# Autodesk Inventor assembly: RP_ROBOT
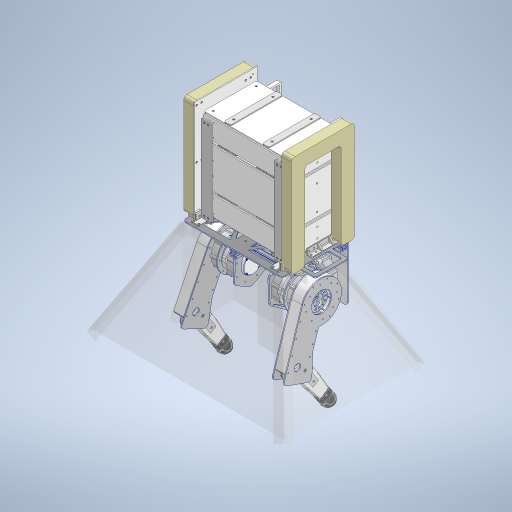
[picture p0: Inventor's stored thumbnail of the model, 512x512]
Saved by Autodesk Inventor 2024.3 (Build 283343000, 343)
## iProperties
Created: 2025-10-10
Part Number: RP_ROBOT
Document SubType Name: Assembly
Designer: 佐藤智貴
Mass: 38781.7 g
Surface Area: 40547 cm^2
Volume: 35004.9 cm^3
Density: 1.10789 g/cm^3
Author: 佐藤智貴
## Documents named in this file (34)
- C:\Users\佐藤智貴\OneDrive - Chiba Institute of Technology\ドキュメント\Inventor\Biped_Robot2\RP_ROBOT.iam
- C:\Users\佐藤智貴\OneDrive - Chiba Institute of Technology\ドキュメント\Inventor\Biped_Robot2\RP_Calf-Foot.ipt
- C:\Users\佐藤智貴\OneDrive - Chiba Institute of Technology\ドキュメント\Inventor\Biped_Robot2\RP_Calf-Link.ipt
- C:\Users\佐藤智貴\OneDrive - Chiba Institute of Technology\ドキュメント\Inventor\Biped_Robot2\RP_Waist-Under-ver2.ipt
- C:\Users\佐藤智貴\OneDrive - Chiba Institute of Technology\ドキュメント\Inventor\Biped_Robot2\RP_Waist-Avobe-ver2.ipt
- C:\Users\佐藤智貴\OneDrive - Chiba Institute of Technology\ドキュメント\Inventor\Biped_Robot2\CAF5-2020-140.ipt
- C:\Users\佐藤智貴\OneDrive - Chiba Institute of Technology\ドキュメント\Inventor\Biped_Robot2\CAF5-2020-170.ipt
- C:\Users\佐藤智貴\OneDrive - Chiba Institute of Technology\ドキュメント\Inventor\Biped_Robot2\CAF5-2020-175.ipt
- C:\Users\佐藤智貴\OneDrive - Chiba Institute of Technology\ドキュメント\Inventor\Biped_Robot2\HFBL45A5-2020-140.iam
- C:\Users\佐藤智貴\OneDrive - Chiba Institute of Technology\ドキュメント\Inventor\Biped_Robot2\8108-8.iam
- C:\Users\佐藤智貴\OneDrive - Chiba Institute of Technology\ドキュメント\Inventor\Biped_Robot2\RP_Hip-Base.ipt
- C:\Users\佐藤智貴\OneDrive - Chiba Institute of Technology\ドキュメント\Inventor\Biped_Robot2\RP_Hip-Link-Left.ipt
- C:\Users\佐藤智貴\OneDrive - Chiba Institute of Technology\ドキュメント\Inventor\Biped_Robot2\RP_Hip-Link-Right.ipt
- C:\Users\佐藤智貴\OneDrive - Chiba Institute of Technology\ドキュメント\Inventor\Biped_Robot2\RP_Calf-Link-cover-Inside-Left.ipt
- C:\Users\佐藤智貴\OneDrive - Chiba Institute of Technology\ドキュメント\Inventor\Biped_Robot2\RP_Calf-Link-cover-Inside-Right.ipt
- C:\Users\佐藤智貴\OneDrive - Chiba Institute of Technology\ドキュメント\Inventor\Biped_Robot2\RP_Calf-Link-cover-Outside-Left.ipt
- C:\Users\佐藤智貴\OneDrive - Chiba Institute of Technology\ドキュメント\Inventor\Biped_Robot2\RP_Calf-Link-cover-Outside-Right.ipt
- C:\Users\佐藤智貴\OneDrive - Chiba Institute of Technology\ドキュメント\Inventor\Biped_Robot2\RP_Thigh-Base_Left.ipt
- C:\Users\佐藤智貴\OneDrive - Chiba Institute of Technology\ドキュメント\Inventor\Biped_Robot2\RP_Thigh-Base-Cover.ipt
- C:\Users\佐藤智貴\OneDrive - Chiba Institute of Technology\ドキュメント\Inventor\Biped_Robot2\RP_Thigh-Base-Right.ipt
- C:\Users\佐藤智貴\OneDrive - Chiba Institute of Technology\ドキュメント\Inventor\Biped_Robot2\RP_Thigh-cover.ipt
- C:\Users\佐藤智貴\OneDrive - Chiba Institute of Technology\ドキュメント\Inventor\Biped_Robot2\RP_Thigh-cover-connect.ipt
- C:\Users\佐藤智貴\OneDrive - Chiba Institute of Technology\ドキュメント\Inventor\Biped_Robot2\RP_Thigh-Link.ipt
- C:\Users\佐藤智貴\OneDrive - Chiba Institute of Technology\ドキュメント\Inventor\Biped_Robot2\simring_34mm.ipt
- C:\Users\佐藤智貴\OneDrive - Chiba Institute of Technology\ドキュメント\Inventor\Biped_Robot2\F688ZZ.ipt
- C:\Users\佐藤智貴\OneDrive - Chiba Institute of Technology\ドキュメント\Inventor\Biped_Robot2\628ZZ.ipt
- C:\Users\佐藤智貴\OneDrive - Chiba Institute of Technology\ドキュメント\Inventor\Biped_Robot2\PSFGW8.ipt
- C:\Users\佐藤智貴\OneDrive - Chiba Institute of Technology\ドキュメント\Inventor\Biped_Robot2\CLBKHM8-20-HC.ipt
- C:\Users\佐藤智貴\OneDrive - Chiba Institute of Technology\ドキュメント\Inventor\Biped_Robot2\RP_Calf-Link-cover-Simring2.5.ipt
- C:\Users\佐藤智貴\OneDrive - Chiba Institute of Technology\ドキュメント\Inventor\Biped_Robot2\RP_Calf-Link-cover-Simring5.5.ipt
- C:\Users\佐藤智貴\OneDrive - Chiba Institute of Technology\ドキュメント\Inventor\Biped_Robot2\RP_Body.iam
- C:\Users\佐藤智貴\OneDrive - Chiba Institute of Technology\ドキュメント\Inventor\Biped_Robot2\RP_Hip-Link-Limit-Long.ipt
- C:\Users\佐藤智貴\OneDrive - Chiba Institute of Technology\ドキュメント\Inventor\Biped_Robot2\RP_Hip-Link-Limit-short.ipt
- C:\Users\佐藤智貴\OneDrive - Chiba Institute of Technology\ドキュメント\Inventor\Biped_Robot2\EX_Assembly.iam
## Components (71 placed, 33 different names)
1. RP_Calf-Foot:1 — メイト:26, 挿入:27
2. RP_Calf-Foot:2 — 挿入:17, メイト:19
3. RP_Calf-Link:1 — 挿入:17, メイト:19, 挿入:18, 挿入:19, 挿入:20, 挿入:21
4. RP_Calf-Link:2 — メイト:26, 挿入:27, 挿入:47, 挿入:48, 挿入:49, 挿入:50
5. RP_Waist-Under-ver2:1 — メイト:1, メイト:2, メイト:3, メイト:4, メイト:5, メイト:6, メイト:7, メイト:8, メイト:15, 挿入:10, 挿入:11, 挿入:15, 挿入:16
6. RP_Waist-Avobe-ver2:1 — メイト:13, メイト:14, メイト:15, 挿入:78, 挿入:79, 挿入:92, 挿入:93
7. CAF5-2020-140:1 — メイト:4, メイト:5, メイト:6, メイト:9, メイト:12, メイト:13
8. CAF5-2020-140:2 — メイト:3, メイト:7, メイト:8, メイト:14
9. CAF5-2020-170:1 — メイト:1, メイト:2, メイト:9, メイト:10, メイト:11, メイト:17
10. CAF5-2020-175:1 — メイト:10, メイト:11, メイト:12, メイト:16, メイト:18
11. HFBL45A5-2020-140:1 [sub-assembly] — メイト:16, メイト:17, メイト:18, メイト:33
12. 8108-8:1 [sub-assembly] — 挿入:5, 挿入:6, 挿入:61, 挿入:62, 挿入:66
13. 8108-8:2 [sub-assembly] — 挿入:1, 挿入:2, 挿入:24, 挿入:25, 挿入:63
14. 8108-8:3 [sub-assembly] — 挿入:14, 挿入:15, 挿入:16, 挿入:80, 挿入:83
15. 8108-8:4 [sub-assembly] — 挿入:3, 挿入:7, 挿入:8, 挿入:84, 挿入:85, 挿入:86, 挿入:87
16. 8108-8:5 [sub-assembly] — 挿入:9, 挿入:10, 挿入:11, 挿入:81, 挿入:82
17. 8108-8:6 [sub-assembly] — 挿入:4, 挿入:12, 挿入:13, 挿入:88, 挿入:89, 挿入:90, 挿入:91
18. RP_Hip-Base:1 — 挿入:1, 挿入:2, 挿入:3
19. RP_Hip-Base:2 — 挿入:4, 挿入:5, 挿入:6
20. RP_Hip-Link-Left:1 — 挿入:12, 挿入:13, 挿入:14
21. RP_Hip-Link-Right:1 — 挿入:7, 挿入:8, 挿入:9
22. RP_Calf-Link-cover-Inside-Left:1 — 挿入:47, 挿入:48, 挿入:53, 挿入:67
23. RP_Calf-Link-cover-Inside-Right:1 — 挿入:18, 挿入:19, 挿入:56, 挿入:64, 挿入:65
24. RP_Calf-Link-cover-Outside-Left:1 — 挿入:49, 挿入:50, 挿入:52, 挿入:54, 挿入:72
25. RP_Calf-Link-cover-Outside-Right:1 — 挿入:20, 挿入:21, 挿入:55, 挿入:71
26. RP_Thigh-Base_Left:1 — 挿入:29, 挿入:30, 挿入:66
27. RP_Thigh-Base-Cover:1 — 挿入:29, 挿入:30, 挿入:51, 挿入:73
28. RP_Thigh-Base-Cover:2 — 挿入:22, 挿入:23, 挿入:70
29. RP_Thigh-Base-Right:1 — 挿入:22, 挿入:23, 挿入:45, 挿入:63
30. RP_Thigh-cover:1 — 挿入:24, 挿入:25, メイト:20, メイト:21, メイト:22, 挿入:65, 挿入:68, 挿入:74
31. RP_Thigh-cover:2 — メイト:23, メイト:24, メイト:25, 挿入:77
32. RP_Thigh-cover:3 — メイト:30, メイト:31, メイト:32, 挿入:76
33. RP_Thigh-cover:4 — メイト:27, メイト:28, メイト:29, 挿入:61, 挿入:62, 挿入:67, 挿入:69, 挿入:75
34. RP_Thigh-cover-connect:1 — メイト:20, メイト:21, メイト:22, メイト:23, メイト:24, メイト:25
35. RP_Thigh-cover-connect:2 — メイト:27, メイト:28, メイト:29, メイト:30, メイト:31, メイト:32
36. RP_Thigh-Link:1 — 挿入:33, 挿入:34, 挿入:37, 挿入:38, 挿入:39, 挿入:40
37. RP_Thigh-Link:2 — 挿入:35, 挿入:36, 挿入:41, 挿入:42, 挿入:43, 挿入:44
38. simring_34mm:1 — 挿入:43, 挿入:51
39. simring_34mm:2 — 挿入:44
40. simring_34mm:3 — 挿入:40
41. simring_34mm:4 — 挿入:42, 挿入:52
42. simring_34mm:5 — 挿入:39, 挿入:45
43. simring_34mm:6 — 挿入:41
44. simring_34mm:7 — 挿入:37
45. simring_34mm:8 — 挿入:38, 挿入:64
46. F688ZZ:1 — 挿入:55
47. F688ZZ:2 — 挿入:53
48. F688ZZ:3 — 挿入:56
49. F688ZZ:4 — 挿入:54
50. 628ZZ:1 — 挿入:33
51. 628ZZ:2 — 挿入:34
52. 628ZZ:3 — 挿入:35
53. 628ZZ:4 — 挿入:36
54. PSFGW8:1 — 挿入:68
55. PSFGW8:2 — 挿入:69
56. CLBKHM8-20-HC:1 — 挿入:71
57. CLBKHM8-20-HC:2 — 挿入:70
58. CLBKHM8-20-HC:3 — 挿入:73
59. CLBKHM8-20-HC:4 — 挿入:72
60. RP_Calf-Link-cover-Simring2.5:1 — 挿入:74
61. RP_Calf-Link-cover-Simring2.5:2 — 挿入:75
62. RP_Calf-Link-cover-Simring5.5:1 — 挿入:77
63. RP_Calf-Link-cover-Simring5.5:2 — 挿入:76
64. RP_Hip-Link-Limit-Long:1 — 挿入:80, 挿入:83
65. RP_Hip-Link-Limit-Long:2 — 挿入:81, 挿入:82
66. RP_Hip-Link-Limit-short:1 — 挿入:88, 挿入:89
67. RP_Hip-Link-Limit-short:2 — 挿入:90, 挿入:91
68. RP_Hip-Link-Limit-short:3 — 挿入:86, 挿入:87
69. RP_Hip-Link-Limit-short:4 — 挿入:84, 挿入:85
70. EX_Assembly:1 [sub-assembly] — 挿入:92, 挿入:93
71. RP_Body:1 [sub-assembly] — 挿入:78, 挿入:79
## Relationships (117: Insert 84, Mate 33)
- メイト:1 [Mate]: RP_Waist-Under-ver2:1 ↔ CAF5-2020-170:1
- メイト:2 [Mate]: RP_Waist-Under-ver2:1 ↔ CAF5-2020-170:1
- メイト:3 [Mate]: RP_Waist-Under-ver2:1 ↔ CAF5-2020-140:2
- メイト:4 [Mate]: RP_Waist-Under-ver2:1 ↔ CAF5-2020-140:1
- メイト:5 [Mate]: RP_Waist-Under-ver2:1 ↔ CAF5-2020-140:1
- メイト:6 [Mate]: RP_Waist-Under-ver2:1 ↔ CAF5-2020-140:1
- メイト:7 [Mate]: RP_Waist-Under-ver2:1 ↔ CAF5-2020-140:2
- メイト:8 [Mate]: RP_Waist-Under-ver2:1 ↔ CAF5-2020-140:2
- メイト:9 [Mate]: CAF5-2020-140:1 ↔ CAF5-2020-170:1
- メイト:10 [Mate]: CAF5-2020-170:1 ↔ CAF5-2020-175:1
- メイト:11 [Mate]: CAF5-2020-170:1 ↔ CAF5-2020-175:1
- メイト:12 [Mate]: CAF5-2020-140:1 ↔ CAF5-2020-175:1
- メイト:13 [Mate]: RP_Waist-Avobe-ver2:1 ↔ CAF5-2020-140:1
- メイト:14 [Mate]: RP_Waist-Avobe-ver2:1 ↔ CAF5-2020-140:2
- メイト:15 [Mate]: RP_Waist-Under-ver2:1 ↔ RP_Waist-Avobe-ver2:1
- メイト:16 [Mate]: CAF5-2020-175:1 ↔ HFBL45A5-2020-140:1
- メイト:17 [Mate]: CAF5-2020-170:1 ↔ HFBL45A5-2020-140:1
- メイト:18 [Mate]: CAF5-2020-175:1 ↔ HFBL45A5-2020-140:1
- 挿入:1 [Insert]: 8108-8:2 ↔ RP_Hip-Base:1
- 挿入:2 [Insert]: 8108-8:2 ↔ RP_Hip-Base:1
- 挿入:3 [Insert]: 8108-8:4 ↔ RP_Hip-Base:1
- 挿入:4 [Insert]: 8108-8:6 ↔ RP_Hip-Base:2
- 挿入:5 [Insert]: 8108-8:1 ↔ RP_Hip-Base:2
- 挿入:6 [Insert]: 8108-8:1 ↔ RP_Hip-Base:2
- 挿入:7 [Insert]: 8108-8:4 ↔ RP_Hip-Link-Right:1
- 挿入:8 [Insert]: 8108-8:4 ↔ RP_Hip-Link-Right:1
- 挿入:9 [Insert]: 8108-8:5 ↔ RP_Hip-Link-Right:1
- 挿入:10 [Insert]: RP_Waist-Under-ver2:1 ↔ 8108-8:5
- 挿入:11 [Insert]: RP_Waist-Under-ver2:1 ↔ 8108-8:5
- 挿入:12 [Insert]: 8108-8:6 ↔ RP_Hip-Link-Left:1
- 挿入:13 [Insert]: 8108-8:6 ↔ RP_Hip-Link-Left:1
- 挿入:14 [Insert]: 8108-8:3 ↔ RP_Hip-Link-Left:1
- 挿入:15 [Insert]: RP_Waist-Under-ver2:1 ↔ 8108-8:3
- 挿入:16 [Insert]: RP_Waist-Under-ver2:1 ↔ 8108-8:3
- 挿入:17 [Insert]: RP_Calf-Foot:2 ↔ RP_Calf-Link:1
- メイト:19 [Mate]: RP_Calf-Foot:2 ↔ RP_Calf-Link:1
- 挿入:18 [Insert]: RP_Calf-Link:1 ↔ RP_Calf-Link-cover-Inside-Right:1
- 挿入:19 [Insert]: RP_Calf-Link:1 ↔ RP_Calf-Link-cover-Inside-Right:1
- 挿入:20 [Insert]: RP_Calf-Link:1 ↔ RP_Calf-Link-cover-Outside-Right:1
- 挿入:21 [Insert]: RP_Calf-Link:1 ↔ RP_Calf-Link-cover-Outside-Right:1
- 挿入:22 [Insert]: RP_Thigh-Base-Cover:2 ↔ RP_Thigh-Base-Right:1
- 挿入:23 [Insert]: RP_Thigh-Base-Cover:2 ↔ RP_Thigh-Base-Right:1
- 挿入:24 [Insert]: 8108-8:2 ↔ RP_Thigh-cover:1
- 挿入:25 [Insert]: 8108-8:2 ↔ RP_Thigh-cover:1
- メイト:20 [Mate]: RP_Thigh-cover:1 ↔ RP_Thigh-cover-connect:1
- メイト:21 [Mate]: RP_Thigh-cover:1 ↔ RP_Thigh-cover-connect:1
- メイト:22 [Mate]: RP_Thigh-cover:1 ↔ RP_Thigh-cover-connect:1
- メイト:23 [Mate]: RP_Thigh-cover:2 ↔ RP_Thigh-cover-connect:1
- メイト:24 [Mate]: RP_Thigh-cover:2 ↔ RP_Thigh-cover-connect:1
- メイト:25 [Mate]: RP_Thigh-cover:2 ↔ RP_Thigh-cover-connect:1
- メイト:26 [Mate]: RP_Calf-Foot:1 ↔ RP_Calf-Link:2
- 挿入:27 [Insert]: RP_Calf-Foot:1 ↔ RP_Calf-Link:2
- 挿入:29 [Insert]: RP_Thigh-Base_Left:1 ↔ RP_Thigh-Base-Cover:1
- 挿入:30 [Insert]: RP_Thigh-Base_Left:1 ↔ RP_Thigh-Base-Cover:1
- メイト:27 [Mate]: RP_Thigh-cover:4 ↔ RP_Thigh-cover-connect:2
- メイト:28 [Mate]: RP_Thigh-cover:4 ↔ RP_Thigh-cover-connect:2
- メイト:29 [Mate]: RP_Thigh-cover:4 ↔ RP_Thigh-cover-connect:2
- メイト:30 [Mate]: RP_Thigh-cover:3 ↔ RP_Thigh-cover-connect:2
- メイト:31 [Mate]: RP_Thigh-cover:3 ↔ RP_Thigh-cover-connect:2
- メイト:32 [Mate]: RP_Thigh-cover:3 ↔ RP_Thigh-cover-connect:2
- 挿入:33 [Insert]: RP_Thigh-Link:1 ↔ 628ZZ:1
- 挿入:34 [Insert]: RP_Thigh-Link:1 ↔ 628ZZ:2
- 挿入:35 [Insert]: RP_Thigh-Link:2 ↔ 628ZZ:3
- 挿入:36 [Insert]: RP_Thigh-Link:2 ↔ 628ZZ:4
- 挿入:37 [Insert]: RP_Thigh-Link:1 ↔ simring_34mm:7
- 挿入:38 [Insert]: RP_Thigh-Link:1 ↔ simring_34mm:8
- 挿入:39 [Insert]: RP_Thigh-Link:1 ↔ simring_34mm:5
- 挿入:40 [Insert]: RP_Thigh-Link:1 ↔ simring_34mm:3
- 挿入:41 [Insert]: RP_Thigh-Link:2 ↔ simring_34mm:6
- 挿入:42 [Insert]: RP_Thigh-Link:2 ↔ simring_34mm:4
- 挿入:43 [Insert]: RP_Thigh-Link:2 ↔ simring_34mm:1
- 挿入:44 [Insert]: RP_Thigh-Link:2 ↔ simring_34mm:2
- 挿入:45 [Insert]: RP_Thigh-Base-Right:1 ↔ simring_34mm:5
- 挿入:47 [Insert]: RP_Calf-Link:2 ↔ RP_Calf-Link-cover-Inside-Left:1
- 挿入:48 [Insert]: RP_Calf-Link:2 ↔ RP_Calf-Link-cover-Inside-Left:1
- 挿入:49 [Insert]: RP_Calf-Link:2 ↔ RP_Calf-Link-cover-Outside-Left:1
- 挿入:50 [Insert]: RP_Calf-Link:2 ↔ RP_Calf-Link-cover-Outside-Left:1
- 挿入:51 [Insert]: RP_Thigh-Base-Cover:1 ↔ simring_34mm:1
- 挿入:52 [Insert]: RP_Calf-Link-cover-Outside-Left:1 ↔ simring_34mm:4
- 挿入:53 [Insert]: RP_Calf-Link-cover-Inside-Left:1 ↔ F688ZZ:2
- 挿入:54 [Insert]: RP_Calf-Link-cover-Outside-Left:1 ↔ F688ZZ:4
- 挿入:55 [Insert]: RP_Calf-Link-cover-Outside-Right:1 ↔ F688ZZ:1
- 挿入:56 [Insert]: RP_Calf-Link-cover-Inside-Right:1 ↔ F688ZZ:3
- 挿入:61 [Insert]: 8108-8:1 ↔ RP_Thigh-cover:4
- 挿入:62 [Insert]: 8108-8:1 ↔ RP_Thigh-cover:4
- 挿入:63 [Insert]: 8108-8:2 ↔ RP_Thigh-Base-Right:1
- 挿入:64 [Insert]: RP_Calf-Link-cover-Inside-Right:1 ↔ simring_34mm:8
- 挿入:65 [Insert] (2.5 mm): RP_Calf-Link-cover-Inside-Right:1 ↔ RP_Thigh-cover:1
- 挿入:66 [Insert]: 8108-8:1 ↔ RP_Thigh-Base_Left:1
- 挿入:67 [Insert] (2.5 mm): RP_Calf-Link-cover-Inside-Left:1 ↔ RP_Thigh-cover:4
- 挿入:68 [Insert]: RP_Thigh-cover:1 ↔ PSFGW8:1
- 挿入:69 [Insert]: RP_Thigh-cover:4 ↔ PSFGW8:2
- 挿入:70 [Insert]: RP_Thigh-Base-Cover:2 ↔ CLBKHM8-20-HC:2
- 挿入:71 [Insert]: RP_Calf-Link-cover-Outside-Right:1 ↔ CLBKHM8-20-HC:1
- 挿入:72 [Insert]: RP_Calf-Link-cover-Outside-Left:1 ↔ CLBKHM8-20-HC:4
- 挿入:73 [Insert]: RP_Thigh-Base-Cover:1 ↔ CLBKHM8-20-HC:3
- 挿入:74 [Insert]: RP_Thigh-cover:1 ↔ RP_Calf-Link-cover-Simring2.5:1
- 挿入:75 [Insert]: RP_Thigh-cover:4 ↔ RP_Calf-Link-cover-Simring2.5:2
- 挿入:76 [Insert]: RP_Thigh-cover:3 ↔ RP_Calf-Link-cover-Simring5.5:2
- 挿入:77 [Insert]: RP_Thigh-cover:2 ↔ RP_Calf-Link-cover-Simring5.5:1
- 挿入:78 [Insert]: RP_Waist-Avobe-ver2:1 ↔ RP_Body:1
- 挿入:79 [Insert]: RP_Waist-Avobe-ver2:1 ↔ RP_Body:1
- メイト:33 [Mate]: HFBL45A5-2020-140:1
- 挿入:80 [Insert]: 8108-8:3 ↔ RP_Hip-Link-Limit-Long:1
- 挿入:81 [Insert]: 8108-8:5 ↔ RP_Hip-Link-Limit-Long:2
- 挿入:82 [Insert]: 8108-8:5 ↔ RP_Hip-Link-Limit-Long:2
- 挿入:83 [Insert]: 8108-8:3 ↔ RP_Hip-Link-Limit-Long:1
- 挿入:84 [Insert]: 8108-8:4 ↔ RP_Hip-Link-Limit-short:4
- 挿入:85 [Insert]: 8108-8:4 ↔ RP_Hip-Link-Limit-short:4
- 挿入:86 [Insert]: 8108-8:4 ↔ RP_Hip-Link-Limit-short:3
- 挿入:87 [Insert]: 8108-8:4 ↔ RP_Hip-Link-Limit-short:3
- 挿入:88 [Insert]: 8108-8:6 ↔ RP_Hip-Link-Limit-short:1
- 挿入:89 [Insert]: 8108-8:6 ↔ RP_Hip-Link-Limit-short:1
- 挿入:90 [Insert]: 8108-8:6 ↔ RP_Hip-Link-Limit-short:2
- 挿入:91 [Insert]: 8108-8:6 ↔ RP_Hip-Link-Limit-short:2
- 挿入:92 [Insert]: RP_Waist-Avobe-ver2:1 ↔ EX_Assembly:1
- 挿入:93 [Insert]: RP_Waist-Avobe-ver2:1 ↔ EX_Assembly:1
